# Autodesk Inventor assembly: STARduino and Pi assembly
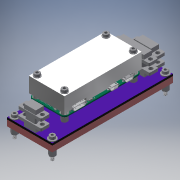
[picture p0: Inventor's stored thumbnail of the model, 180x180]
Saved by Autodesk Inventor 2017 (Build 210142000, 142)
## iProperties
Created: 2017-01-16
Part Number: STARduino and Pi assembly
Document SubType Name: Assembly
Designer: qupec
Mass: 94.0986 g
Surface Area: 327.317 cm^2
Volume: 52.2385 cm^3
Density: 1.80133 g/cm^3
Author: qupec
## Documents named in this file (16)
- C:\UMD\BPP\ROCKSAT X\STAR\CAD\Mechanical\Full payload assembly\Subsystems\Electronics\Electronics Stack.iam
- C:\UMD\BPP\ROCKSAT X\STAR\CAD\Mechanical\Full payload assembly\Subsystems\Electronics\STARduino.ipt
- C:\UMD\BPP\ROCKSAT X\STAR\CAD\Mechanical\Full payload assembly\Subsystems\Electronics\STARduino Mat.ipt
- C:\UMD\BPP\ROCKSAT X\STAR\CAD\Mechanical\Full payload assembly\Subsystems\Electronics\Raspberry Pi.ipt
- C:\UMD\BPP\ROCKSAT X\STAR\CAD\Mechanical\Full payload assembly\Subsystems\Electronics\Heat Block.ipt
- C:\UMD\BPP\ROCKSAT X\STAR\CAD\Mechanical\Full payload assembly\Subsystems\Electronics\31pin female connector.ipt
- C:\UMD\BPP\ROCKSAT X\STAR\CAD\Mechanical\Full payload assembly\Subsystems\Electronics\15pin female connector.ipt
- C:\UMD\BPP\ROCKSAT X\STAR\CAD\Mechanical\Full payload assembly\Subsystems\Electronics\9pin female connector.ipt
- C:\UMD\BPP\ROCKSAT X\STAR\CAD\Mechanical\Full payload assembly\Subsystems\Electronics\31pin male connector.ipt
- C:\UMD\BPP\ROCKSAT X\STAR\CAD\Mechanical\Full payload assembly\Subsystems\Electronics\15pin male connector.ipt
- C:\UMD\BPP\ROCKSAT X\STAR\CAD\Mechanical\Full payload assembly\Subsystems\Electronics\9pin male connector.ipt
- C:\UMD\BPP\ROCKSAT X\STAR\CAD\Mechanical\Full payload assembly\Subsystems\Fasteners\M2.5 5mm Standoff.ipt
- C:\UMD\BPP\ROCKSAT X\STAR\CAD\Mechanical\Full payload assembly\Subsystems\Fasteners\M2.5 Insulating Washer.ipt
- C:\UMD\BPP\ROCKSAT X\STAR\CAD\Mechanical\Full payload assembly\Subsystems\Fasteners\M2.5 5mm Socket Screw.ipt
- C:\UMD\BPP\ROCKSAT X\STAR\CAD\Mechanical\Full payload assembly\Subsystems\Fasteners\M2.5 Tooth Washer.ipt
- C:\UMD\BPP\ROCKSAT X\STAR\CAD\Mechanical\Full payload assembly\Subsystems\Fasteners\M2.5x.45mm 20mm Socket Screw.ipt
## Components (38 placed, 15 different names)
1. STARduino:1 — Mate:7, Mate:23, Mate:24, Mate:32, Mate:33, Mate:34, Flush:1, Flush:3, Flush:4, Flush:5, Flush:6, Flush:7, Mate:54, Mate:55, Mate:56, Mate:57, Mate:58, Mate:59, Mate:60, Mate:61, Mate:62, Mate:67, Mate:73, Mate:74, Mate:75, Mate:76, Mate:85, Mate:86, Mate:87, Mate:88
2. STARduino Mat:1 — Mate:7, Mate:23, Mate:24, Mate:44, Mate:45, Flush:8, Mate:46, Mate:47, Mate:48, Mate:49, Mate:50, Mate:51, Mate:52, Mate:53, Mate:68, Mate:69, Mate:77, Mate:78, Mate:79, Mate:80
3. Raspberry Pi:1 — Mate:26, Mate:27, Mate:28, Mate:70
4. Heat Block:1 — Mate:26, Mate:27, Mate:28, Mate:71, Mate:72, Mate:89, Mate:90, Mate:91, Mate:92, Mate:93, Mate:94, Mate:95, Mate:96, Mate:97, Mate:98, Mate:99, Mate:100, Mate:101, Mate:102, Mate:103, Mate:104
5. 31pin female connector:1 — Mate:34, Flush:3, Flush:5, Mate:35, Mate:40, Mate:41
6. 15pin female connector:1 — Mate:33, Mate:36, Mate:39, Mate:42, Flush:6, Flush:7
7. 9pin female connector:1 — Mate:32, Flush:1, Flush:4, Mate:37, Mate:38, Mate:43
8. 31pin male connector:1 — Mate:35, Mate:40, Mate:41
9. 15pin male connector:1 — Mate:36, Mate:39, Mate:42
10. 9pin male connector:1 — Mate:37, Mate:38, Mate:43
11. M2.5 5mm Standoff:1 — Mate:57, Mate:58, Mate:66, Mate:72
12. M2.5 5mm Standoff:2 — Mate:56, Mate:61, Mate:64, Mate:70, Mate:71
13. M2.5 5mm Standoff:3 — Mate:55, Mate:59, Mate:65
14. M2.5 5mm Standoff:4 — Mate:54, Mate:60, Mate:63
15. M2.5 5mm Standoff:5 — Mate:49, Mate:69
16. M2.5 5mm Standoff:6 — Mate:50, Mate:65
17. M2.5 5mm Standoff:7 — Mate:51, Mate:68
18. M2.5 5mm Standoff:8 — Mate:52, Mate:67
19. M2.5 5mm Standoff:9 — Mate:46, Mate:66
20. M2.5 5mm Standoff:10 — Mate:47, Mate:63
21. M2.5 5mm Standoff:11 — Mate:48, Mate:64
22. M2.5 5mm Standoff:12 — Mate:53, Mate:62
23. M2.5 Insulating Washer:1 — Mate:73, Mate:77, Mate:81
24. M2.5 Insulating Washer:2 — Mate:74, Mate:78, Mate:82
25. M2.5 Insulating Washer:3 — Mate:75, Mate:79, Mate:84
26. M2.5 Insulating Washer:4 — Mate:76, Mate:80, Mate:83
27. M2.5 5mm Socket Screw:1 — Mate:81, Mate:88
28. M2.5 5mm Socket Screw:2 — Mate:82, Mate:87
29. M2.5 5mm Socket Screw:3 — Mate:83, Mate:85
30. M2.5 5mm Socket Screw:4 — Mate:84, Mate:86
31. M2.5 Tooth Washer:1 — Mate:91, Mate:95
32. M2.5 Tooth Washer:2 — Mate:92, Mate:96
33. M2.5 Tooth Washer:3 — Mate:90, Mate:94
34. M2.5 Tooth Washer:4 — Mate:89, Mate:93
35. M2.5x.45mm 20mm Socket Screw:1 — Mate:97, Mate:101
36. M2.5x.45mm 20mm Socket Screw:2 — Mate:98, Mate:103
37. M2.5x.45mm 20mm Socket Screw:3 — Mate:99, Mate:102
38. M2.5x.45mm 20mm Socket Screw:4 — Mate:100, Mate:104
## Relationships (86: Mate 79, Flush 7)
- Mate:7: STARduino:1 ↔ STARduino Mat:1
- Mate:23: STARduino:1 ↔ STARduino Mat:1
- Mate:24: STARduino:1 ↔ STARduino Mat:1
- Mate:26: Raspberry Pi:1 ↔ Heat Block:1
- Mate:27: Raspberry Pi:1 ↔ Heat Block:1
- Mate:28: Raspberry Pi:1 ↔ Heat Block:1
- Mate:32: STARduino:1 ↔ 9pin female connector:1
- Mate:33: STARduino:1 ↔ 15pin female connector:1
- Mate:34: STARduino:1 ↔ 31pin female connector:1
- Flush:1: STARduino:1 ↔ 9pin female connector:1
- Flush:3 (7.62 mm): STARduino:1 ↔ 31pin female connector:1
- Flush:4 (8.89 mm): STARduino:1 ↔ 9pin female connector:1
- Flush:5: STARduino:1 ↔ 31pin female connector:1
- Mate:35: 31pin female connector:1 ↔ 31pin male connector:1
- Mate:36: 15pin female connector:1 ↔ 15pin male connector:1
- Mate:37: 9pin female connector:1 ↔ 9pin male connector:1
- Mate:38: 9pin female connector:1 ↔ 9pin male connector:1
- Mate:39: 15pin female connector:1 ↔ 15pin male connector:1
- Mate:40: 31pin female connector:1 ↔ 31pin male connector:1
- Mate:41: 31pin female connector:1 ↔ 31pin male connector:1
- Mate:42: 15pin female connector:1 ↔ 15pin male connector:1
- Mate:43: 9pin female connector:1 ↔ 9pin male connector:1
- Flush:6: STARduino:1 ↔ 15pin female connector:1
- Flush:7 (6.35 mm): STARduino:1 ↔ 15pin female connector:1
- Mate:44: STARduino Mat:1
- Mate:45: STARduino Mat:1
- Flush:8: STARduino Mat:1
- Mate:46: STARduino Mat:1 ↔ M2.5 5mm Standoff:9
- Mate:47: STARduino Mat:1 ↔ M2.5 5mm Standoff:10
- Mate:48: STARduino Mat:1 ↔ M2.5 5mm Standoff:11
- Mate:49: STARduino Mat:1 ↔ M2.5 5mm Standoff:5
- Mate:50: STARduino Mat:1 ↔ M2.5 5mm Standoff:6
- Mate:51: STARduino Mat:1 ↔ M2.5 5mm Standoff:7
- Mate:52: STARduino Mat:1 ↔ M2.5 5mm Standoff:8
- Mate:53: STARduino Mat:1 ↔ M2.5 5mm Standoff:12
- Mate:54: STARduino:1 ↔ M2.5 5mm Standoff:4
- Mate:55: STARduino:1 ↔ M2.5 5mm Standoff:3
- Mate:56: STARduino:1 ↔ M2.5 5mm Standoff:2
- Mate:57: STARduino:1 ↔ M2.5 5mm Standoff:1
- Mate:58: STARduino:1 ↔ M2.5 5mm Standoff:1
- Mate:59: STARduino:1 ↔ M2.5 5mm Standoff:3
- Mate:60: STARduino:1 ↔ M2.5 5mm Standoff:4
- Mate:61: STARduino:1 ↔ M2.5 5mm Standoff:2
- Mate:62: STARduino:1 ↔ M2.5 5mm Standoff:12
- Mate:63: M2.5 5mm Standoff:4 ↔ M2.5 5mm Standoff:10
- Mate:64: M2.5 5mm Standoff:2 ↔ M2.5 5mm Standoff:11
- Mate:65: M2.5 5mm Standoff:3 ↔ M2.5 5mm Standoff:6
- Mate:66: M2.5 5mm Standoff:1 ↔ M2.5 5mm Standoff:9
- Mate:67: STARduino:1 ↔ M2.5 5mm Standoff:8
- Mate:68: STARduino Mat:1 ↔ M2.5 5mm Standoff:7
- Mate:69: STARduino Mat:1 ↔ M2.5 5mm Standoff:5
- Mate:70: Raspberry Pi:1 ↔ M2.5 5mm Standoff:2
- Mate:71: Heat Block:1 ↔ M2.5 5mm Standoff:2
- Mate:72: Heat Block:1 ↔ M2.5 5mm Standoff:1
- Mate:73: STARduino:1 ↔ M2.5 Insulating Washer:1
- Mate:74: STARduino:1 ↔ M2.5 Insulating Washer:2
- Mate:75: STARduino:1 ↔ M2.5 Insulating Washer:3
- Mate:76: STARduino:1 ↔ M2.5 Insulating Washer:4
- Mate:77: STARduino Mat:1 ↔ M2.5 Insulating Washer:1
- Mate:78: STARduino Mat:1 ↔ M2.5 Insulating Washer:2
- Mate:79: STARduino Mat:1 ↔ M2.5 Insulating Washer:3
- Mate:80: STARduino Mat:1 ↔ M2.5 Insulating Washer:4
- Mate:81: M2.5 Insulating Washer:1 ↔ M2.5 5mm Socket Screw:1
- Mate:82: M2.5 Insulating Washer:2 ↔ M2.5 5mm Socket Screw:2
- Mate:83: M2.5 Insulating Washer:4 ↔ M2.5 5mm Socket Screw:3
- Mate:84: M2.5 Insulating Washer:3 ↔ M2.5 5mm Socket Screw:4
- Mate:85: STARduino:1 ↔ M2.5 5mm Socket Screw:3
- Mate:86: STARduino:1 ↔ M2.5 5mm Socket Screw:4
- Mate:87: STARduino:1 ↔ M2.5 5mm Socket Screw:2
- Mate:88: STARduino:1 ↔ M2.5 5mm Socket Screw:1
- Mate:89: Heat Block:1 ↔ M2.5 Tooth Washer:4
- Mate:90: Heat Block:1 ↔ M2.5 Tooth Washer:3
- Mate:91: Heat Block:1 ↔ M2.5 Tooth Washer:1
- Mate:92: Heat Block:1 ↔ M2.5 Tooth Washer:2
- Mate:93: Heat Block:1 ↔ M2.5 Tooth Washer:4
- Mate:94: Heat Block:1 ↔ M2.5 Tooth Washer:3
- Mate:95: Heat Block:1 ↔ M2.5 Tooth Washer:1
- Mate:96: Heat Block:1 ↔ M2.5 Tooth Washer:2
- Mate:97: Heat Block:1 ↔ M2.5x.45mm 20mm Socket Screw:1
- Mate:98: Heat Block:1 ↔ M2.5x.45mm 20mm Socket Screw:2
- Mate:99: Heat Block:1 ↔ M2.5x.45mm 20mm Socket Screw:3
- Mate:100: Heat Block:1 ↔ M2.5x.45mm 20mm Socket Screw:4
- Mate:101: Heat Block:1 ↔ M2.5x.45mm 20mm Socket Screw:1
- Mate:102: Heat Block:1 ↔ M2.5x.45mm 20mm Socket Screw:3
- Mate:103: Heat Block:1 ↔ M2.5x.45mm 20mm Socket Screw:2
- Mate:104: Heat Block:1 ↔ M2.5x.45mm 20mm Socket Screw:4
